# Autodesk Inventor assembly: MQ Exploded View
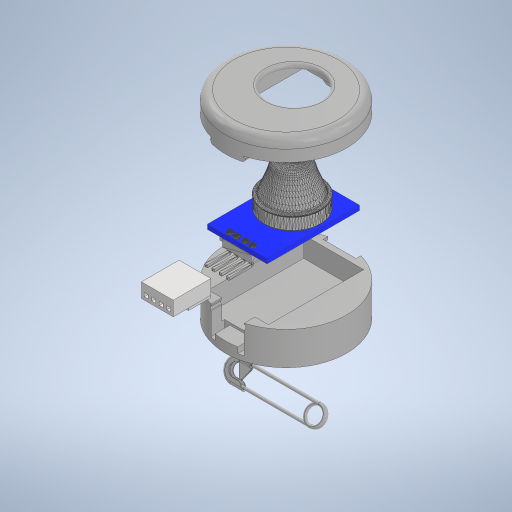
[picture p0: Inventor's stored thumbnail of the model, 512x512]
Saved by Autodesk Inventor 2023 (Build 270158000, 158)
## iProperties
Created: 2024-03-19
Part Number: MQ Exploded View
Document SubType Name: Assembly
Designer: ongyu
Author: ongyu
## Documents named in this file (6)
- C:\Users\ongyu\OneDrive\Documents\Inventor\FYP\MQ-Shell\MQ-Exploded-View.iam
- C:\Users\ongyu\OneDrive\Documents\Inventor\FYP\MQ-Shell\01 - MQ-Case-Btm.ipt
- C:\Users\ongyu\OneDrive\Documents\Inventor\FYP\MQ-Shell\02 - MQ-Case-Top.ipt
- C:\Users\ongyu\OneDrive\Documents\Inventor\FYP\MQ-Shell\03 - MQ.ipt
- C:\Users\ongyu\OneDrive\Documents\Inventor\FYP\MQ-Shell\04 - Four-Pin-Connector.ipt
- C:\Users\ongyu\OneDrive\Documents\Inventor\FYP\MQ-Shell\05 - Safety-Pin.ipt
## Components (5 placed, 5 different names)
1. 01 - MQ-Case-Btm:1 — Flush:1, Mate:1, Flush:2, Mate:4, Mate:5, Insert:1
2. 02 - MQ-Case-Top:1 — Insert:1
3. 03 - MQ:1 — Mate:4, Mate:5, Mate:7, Mate:8, Flush:3
4. 04 - Four-Pin-Connector:1 — Mate:8, Flush:3
5. 05 - Safety-Pin:1 — Flush:4, Flush:5
## Relationships (11: Flush 5, Mate 5, Insert 1)
- Flush:1: 01 - MQ-Case-Btm:1
- Mate:1: 01 - MQ-Case-Btm:1
- Flush:2: 01 - MQ-Case-Btm:1
- Mate:4: 01 - MQ-Case-Btm:1 ↔ 03 - MQ:1
- Mate:5 (25 mm): 01 - MQ-Case-Btm:1 ↔ 03 - MQ:1
- Insert:1 (50 mm): 01 - MQ-Case-Btm:1 ↔ 02 - MQ-Case-Top:1
- Mate:7: 03 - MQ:1
- Mate:8: 03 - MQ:1 ↔ 04 - Four-Pin-Connector:1
- Flush:3: 03 - MQ:1 ↔ 04 - Four-Pin-Connector:1
- Flush:4 (15 mm): 05 - Safety-Pin:1
- Flush:5: 05 - Safety-Pin:1
